# Autodesk Inventor assembly: Pipe System Assembly
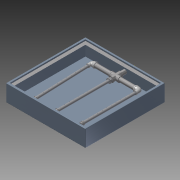
[picture p0: Inventor's stored thumbnail of the model, 180x180]
Saved by Autodesk Inventor 2013 SP2 (Build 170200200, 200)
## iProperties
Created: 2014-05-30
Part Number: Pipe System Assembly
Document SubType Name: Assembly
Designer: jmw3
Author: jmw3
## Documents named in this file (9)
- F:\NIST\Propane Burner\Pipe System Assembly.iam
- F:\NIST\Propane Burner\Propane Burner Base.ipt
- F:\NIST\Propane Burner\Cross Pipe Fitting ASME B16.3 Class 150.ipt
- F:\NIST\Propane Burner\Welded Pipe Fitting ASTM A312 Schedule 40.ipt
- F:\NIST\Propane Burner\1 in pipe ASTM A 312 - Schedule 40S.ipt
- F:\NIST\Propane Burner\.5 in pipe.ipt
- F:\NIST\Propane Burner\.5 in pipe cap.ipt
- F:\NIST\Propane Burner\1 in to .5 in elbow reducer.ipt
- F:\NIST\Propane Burner\1 in to .5 in reducer.ipt
## Components (14 placed, 8 different names)
1. Propane Burner Base:1 — Mate:4, Flush:1, Rotation:1, Mate:44, Mate:45
2. Cross Pipe Fitting ASME B16.3 Class 150:1 — Mate:5, Mate:6, Rotation:2, Mate:7, Mate:8, Rotation:3, Mate:28, Mate:29, Rotation:13, Mate:51, Mate:52
3. Welded Pipe Fitting ASTM A312 Schedule 40:1 — Mate:4, Flush:1, Rotation:1, Mate:5, Mate:6, Rotation:2, Mate:44, Mate:45
4. 1 in pipe ASTM A 312 - Schedule 40S:1 — Mate:7, Mate:8, Rotation:3, Mate:48, Mate:49, Mate:50, Rotation:21
5. .5 in pipe cap:1 — Mate:58, Mate:59
6. 1 in pipe ASTM A 312 - Schedule 40S:2 — Mate:28, Mate:29, Rotation:13, Mate:46, Mate:47, Insert:1, Rotation:20
7. .5 in pipe cap:4 — Mate:55, Mate:56
8. .5 in pipe cap:5 — Mate:61, Flush:4
9. 1 in to .5 in elbow reducer:1 — Mate:48, Mate:49, Mate:50, Rotation:21, Mate:57, Flush:2
10. 1 in to .5 in elbow reducer:2 — Mate:46, Mate:47, Insert:1, Rotation:20, Mate:60, Flush:3
11. .5 in pipe:1 — Mate:60, Flush:3, Mate:61, Flush:4
12. .5 in pipe:2 — Mate:57, Flush:2, Mate:58, Mate:59
13. .5 in pipe:3 — Mate:53, Mate:54, Mate:55, Mate:56
14. 1 in to .5 in reducer:1 — Mate:51, Mate:52, Mate:53, Mate:54
## Relationships (36: Mate 25, RelateRotation 6, Flush 4, Insert 1)
- Mate:4: Propane Burner Base:1 ↔ Welded Pipe Fitting ASTM A312 Schedule 40:1
- Flush:1 (-25.4 mm): Propane Burner Base:1 ↔ Welded Pipe Fitting ASTM A312 Schedule 40:1
- Rotation:1 [RelateRotation] (1 ul): Propane Burner Base:1 ↔ Welded Pipe Fitting ASTM A312 Schedule 40:1
- Mate:5: Cross Pipe Fitting ASME B16.3 Class 150:1 ↔ Welded Pipe Fitting ASTM A312 Schedule 40:1
- Mate:6: Cross Pipe Fitting ASME B16.3 Class 150:1 ↔ Welded Pipe Fitting ASTM A312 Schedule 40:1
- Rotation:2 [RelateRotation] (1 ul): Cross Pipe Fitting ASME B16.3 Class 150:1 ↔ Welded Pipe Fitting ASTM A312 Schedule 40:1
- Mate:7: Cross Pipe Fitting ASME B16.3 Class 150:1 ↔ 1 in pipe ASTM A 312 - Schedule 40S:1
- Mate:8: Cross Pipe Fitting ASME B16.3 Class 150:1 ↔ 1 in pipe ASTM A 312 - Schedule 40S:1
- Rotation:3 [RelateRotation] (1 ul): Cross Pipe Fitting ASME B16.3 Class 150:1 ↔ 1 in pipe ASTM A 312 - Schedule 40S:1
- Mate:28: Cross Pipe Fitting ASME B16.3 Class 150:1 ↔ 1 in pipe ASTM A 312 - Schedule 40S:2
- Mate:29: Cross Pipe Fitting ASME B16.3 Class 150:1 ↔ 1 in pipe ASTM A 312 - Schedule 40S:2
- Rotation:13 [RelateRotation] (0.743 ul): Cross Pipe Fitting ASME B16.3 Class 150:1 ↔ 1 in pipe ASTM A 312 - Schedule 40S:2
- Mate:44: Propane Burner Base:1 ↔ Welded Pipe Fitting ASTM A312 Schedule 40:1
- Mate:45: Propane Burner Base:1 ↔ Welded Pipe Fitting ASTM A312 Schedule 40:1
- Mate:46: 1 in pipe ASTM A 312 - Schedule 40S:2 ↔ 1 in to .5 in elbow reducer:2
- Mate:47: 1 in pipe ASTM A 312 - Schedule 40S:2 ↔ 1 in to .5 in elbow reducer:2
- Insert:1: 1 in pipe ASTM A 312 - Schedule 40S:2 ↔ 1 in to .5 in elbow reducer:2
- Rotation:20 [RelateRotation] (0.593 ul): 1 in pipe ASTM A 312 - Schedule 40S:2 ↔ 1 in to .5 in elbow reducer:2
- Mate:48: 1 in pipe ASTM A 312 - Schedule 40S:1 ↔ 1 in to .5 in elbow reducer:1
- Mate:49: 1 in pipe ASTM A 312 - Schedule 40S:1 ↔ 1 in to .5 in elbow reducer:1
- Mate:50: 1 in pipe ASTM A 312 - Schedule 40S:1 ↔ 1 in to .5 in elbow reducer:1
- Mate:51: Cross Pipe Fitting ASME B16.3 Class 150:1 ↔ 1 in to .5 in reducer:1
- Mate:52: Cross Pipe Fitting ASME B16.3 Class 150:1 ↔ 1 in to .5 in reducer:1
- Mate:53: .5 in pipe:3 ↔ 1 in to .5 in reducer:1
- Mate:54: .5 in pipe:3 ↔ 1 in to .5 in reducer:1
- Mate:55: .5 in pipe cap:4 ↔ .5 in pipe:3
- Mate:56: .5 in pipe cap:4 ↔ .5 in pipe:3
- Rotation:21 [RelateRotation] (1 ul): 1 in pipe ASTM A 312 - Schedule 40S:1 ↔ 1 in to .5 in elbow reducer:1
- Mate:57: 1 in to .5 in elbow reducer:1 ↔ .5 in pipe:2
- Flush:2: 1 in to .5 in elbow reducer:1 ↔ .5 in pipe:2
- Mate:58: .5 in pipe cap:1 ↔ .5 in pipe:2
- Mate:59: .5 in pipe cap:1 ↔ .5 in pipe:2
- Mate:60: 1 in to .5 in elbow reducer:2 ↔ .5 in pipe:1
- Flush:3: 1 in to .5 in elbow reducer:2 ↔ .5 in pipe:1
- Mate:61: .5 in pipe cap:5 ↔ .5 in pipe:1
- Flush:4: .5 in pipe cap:5 ↔ .5 in pipe:1
